# Autodesk Inventor assembly: Hose Clamp
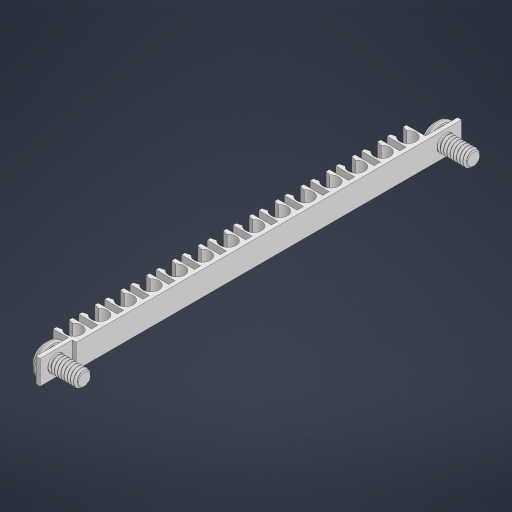
[picture p0: Inventor's stored thumbnail of the model, 512x512]
Saved by Autodesk Inventor 2024 (Build 280153000, 153)
## iProperties
Created: 2023-05-24
Part Number: Hose Clamp
Document SubType Name: Assembly
Designer: cfangmeier3
Author: cfangmeier3
## Documents named in this file (3)
- C:\Users\cfangmeier3\Desktop\nebraska-silicon-lab\Hardware\General Gantry\Hose Clamp\Hose Clamp.iam
- C:\Users\cfangmeier3\Desktop\nebraska-silicon-lab\Hardware\General Gantry\Hose Clamp\Hose Clamp.ipt
- C:\Users\cfangmeier3\Desktop\nebraska-silicon-lab\Hardware\General Gantry\Hose Clamp\91772A537_Passivated 18-8 Stainless Steel Pan Head Phillips Screw\91772A537_Passivated 18-8 Stainless Steel Pan Head Phillips.ipt
## Components (3 placed, 2 different names)
1. Hose Clamp:1 — Insert:1, Insert:2
2. 91772A537_Passivated 18-8 Stainless Steel Pan Head Phillips:1 — Insert:1
3. 91772A537_Passivated 18-8 Stainless Steel Pan Head Phillips:2 — Insert:2
## Relationships (2: Insert 2)
- Insert:1: Hose Clamp:1 ↔ 91772A537_Passivated 18-8 Stainless Steel Pan Head Phillips:1
- Insert:2: Hose Clamp:1 ↔ 91772A537_Passivated 18-8 Stainless Steel Pan Head Phillips:2
